# Autodesk Inventor assembly: YaxisAss
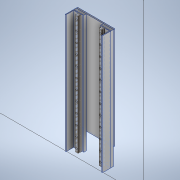
[picture p0: Inventor's stored thumbnail of the model, 180x180]
Saved by Autodesk Inventor 2022 (Build 260153000, 153)
## iProperties
Created: 2023-08-15
Part Number: YaxisAss
Document SubType Name: Assembly
Designer: Kippi
Mass: 8048.7 g
Surface Area: 7726.2 cm^2
Volume: 2981 cm^3
Density: 2.7 g/cm^3
Author: Kippi
## Documents named in this file (5)
- C:\Users\Kippi\Documents\CNC_Lathe\YaxisAss.iam
- C:\Users\Kippi\Documents\CNC_Lathe\PodkladkaY.ipt
- C:\Users\Kippi\Documents\CNC_Lathe\Ugol700.ipt
- C:\Users\Kippi\Documents\CNC_Lathe\AxisY.ipt
- C:\Users\Kippi\Documents\CNC_Lathe\Rails\HGR20R LINEAR GUIDE RAIL, CONFIGURABLE, 700 mm.ipt
## Components (7 placed, 4 different names)
1. PodkladkaY:1 — Mate:1, Flush:3, Flush:4, Mate:3, Flush:6, Flush:11
2. Ugol700:1 — Mate:3, Flush:5, Flush:6, Mate:6, Flush:10
3. PodkladkaY:2 — Mate:2, Flush:1, Flush:2, Mate:4, Flush:7, Flush:8, Flush:12
4. Ugol700:2 — Mate:4, Flush:7, Flush:8, Mate:5, Flush:9
5. AxisY:1 — Mate:1, Mate:2, Flush:1, Flush:2, Flush:3, Flush:4, Flush:5
6. HGR20R LINEAR GUIDE RAIL, CONFIGURABLE, 700 mm:1 — Mate:5, Flush:9, Flush:12
7. HGR20R LINEAR GUIDE RAIL, CONFIGURABLE, 700 mm:2 — Mate:6, Flush:10, Flush:11
## Relationships (18: Flush 12, Mate 6)
- Mate:1: PodkladkaY:1 ↔ AxisY:1
- Mate:2: PodkladkaY:2 ↔ AxisY:1
- Flush:1: PodkladkaY:2 ↔ AxisY:1
- Flush:2: PodkladkaY:2 ↔ AxisY:1
- Flush:3: PodkladkaY:1 ↔ AxisY:1
- Flush:4: PodkladkaY:1 ↔ AxisY:1
- Mate:3: PodkladkaY:1 ↔ Ugol700:1
- Flush:5: Ugol700:1 ↔ AxisY:1
- Flush:6: PodkladkaY:1 ↔ Ugol700:1
- Mate:4: PodkladkaY:2 ↔ Ugol700:2
- Flush:7: PodkladkaY:2 ↔ Ugol700:2
- Flush:8: PodkladkaY:2 ↔ Ugol700:2
- Mate:5: Ugol700:2 ↔ HGR20R LINEAR GUIDE RAIL, CONFIGURABLE, 700 mm:1
- Mate:6: Ugol700:1 ↔ HGR20R LINEAR GUIDE RAIL, CONFIGURABLE, 700 mm:2
- Flush:9: Ugol700:2 ↔ HGR20R LINEAR GUIDE RAIL, CONFIGURABLE, 700 mm:1
- Flush:10: Ugol700:1 ↔ HGR20R LINEAR GUIDE RAIL, CONFIGURABLE, 700 mm:2
- Flush:11: PodkladkaY:1 ↔ HGR20R LINEAR GUIDE RAIL, CONFIGURABLE, 700 mm:2
- Flush:12: PodkladkaY:2 ↔ HGR20R LINEAR GUIDE RAIL, CONFIGURABLE, 700 mm:1
